# Autodesk Inventor assembly: Assembly
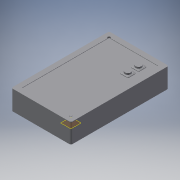
[picture p0: Inventor's stored thumbnail of the model, 180x180]
Saved by Autodesk Inventor 2019 (Build 230136000, 136)
## iProperties
Created: 2018-10-23
Part Number: Assembly
Document SubType Name: Assembly
Designer: Administrator
Author: Administrator
## Documents named in this file (4)
- C:\Users\Administrator\Downloads\Video Switch Box\Assembly.iam
- C:\Users\Administrator\Downloads\Video Switch Box\Box.ipt
- C:\Users\Administrator\Downloads\Video Switch Box\Lid.ipt
- C:\Users\Administrator\Downloads\Video Switch Box\Switch.ipt
## Components (4 placed, 3 different names)
1. Box:1 — Flush:1, Flush:2, Mate:1
2. Lid:1 — Flush:1, Flush:2, Mate:1, Mate:2, Mate:3, Mate:4, Mate:5
3. Switch:1 — Mate:2, Mate:4
4. Switch:2 — Mate:3, Mate:5
## Relationships (7: Mate 5, Flush 2)
- Flush:1: Box:1 ↔ Lid:1
- Flush:2: Box:1 ↔ Lid:1
- Mate:1: Box:1 ↔ Lid:1
- Mate:2: Lid:1 ↔ Switch:1
- Mate:3: Lid:1 ↔ Switch:2
- Mate:4: Lid:1 ↔ Switch:1
- Mate:5: Lid:1 ↔ Switch:2
